# Autodesk Inventor assembly: TruckWithMotors
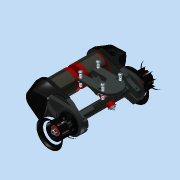
[picture p0: Inventor's stored thumbnail of the model, 180x180]
Saved by Autodesk Inventor 2015 (Build 190159000, 159)
## iProperties
Created: 2015-11-06
Part Number: TruckWithMotors
Document SubType Name: Assembly
Designer: Raphael
Author: Raphael
## Documents named in this file (5)
- \\psf\Home\Documents\electric-skateboard\CAD\TruckWithMotors.iam
- \\psf\Home\Documents\electric-skateboard\CAD\MotorMount.iam
- \\psf\Home\Documents\electric-skateboard\CAD\ParisTruck.iam
- \\psf\Home\Documents\electric-skateboard\CAD\WheelWithPulley.iam
- \\psf\Home\Documents\electric-skateboard\CAD\Belt.ipt
## Components (7 placed, 4 different names)
1. MotorMount:1 [sub-assembly] — Mate:5, Mate:8, Mate:10, Tangent:1, Mate:13
2. MotorMount:2 [sub-assembly] — Mate:6, Mate:10, Mate:11, Mate:15
3. ParisTruck:1 [sub-assembly] — Mate:1, Mate:3, Mate:4, Mate:5, Mate:6, Mate:9, Tangent:1
4. WheelWithPulley:1 [sub-assembly] — Mate:1, Mate:4, Mate:8, Mate:12, Flush:1
5. WheelWithPulley:2 [sub-assembly] — Mate:3, Mate:9, Mate:11, Mate:14, Flush:2
6. Belt:1 — Mate:12, Mate:13, Flush:1
7. Belt:2 — Mate:14, Mate:15, Flush:2
## Relationships (16: Mate 13, Flush 2, Tangent 1)
- Mate:1: ParisTruck:1 ↔ WheelWithPulley:1
- Mate:3 (1 mm): ParisTruck:1 ↔ WheelWithPulley:2
- Mate:4 (1 mm): ParisTruck:1 ↔ WheelWithPulley:1
- Mate:5: MotorMount:1 ↔ ParisTruck:1
- Mate:6: MotorMount:2 ↔ ParisTruck:1
- Mate:8 (0.5 mm): MotorMount:1 ↔ WheelWithPulley:1
- Mate:9: ParisTruck:1 ↔ WheelWithPulley:2
- Mate:10: MotorMount:1 ↔ MotorMount:2
- Mate:11: MotorMount:2 ↔ WheelWithPulley:2
- Tangent:1 (3 mm): MotorMount:1 ↔ ParisTruck:1
- Mate:12: WheelWithPulley:1 ↔ Belt:1
- Mate:13: MotorMount:1 ↔ Belt:1
- Flush:1: WheelWithPulley:1 ↔ Belt:1
- Mate:14: WheelWithPulley:2 ↔ Belt:2
- Mate:15: MotorMount:2 ↔ Belt:2
- Flush:2: WheelWithPulley:2 ↔ Belt:2
